# Autodesk Inventor assembly: Marco_triciclo
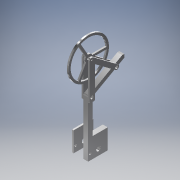
[picture p0: Inventor's stored thumbnail of the model, 180x180]
Saved by Autodesk Inventor 2019 (Build 230136000, 136)
## iProperties
Created: 2019-11-14
Part Number: Marco_triciclo
Document SubType Name: Assembly
Designer: Domenico
Mass: 2567.25 g
Surface Area: 2052.12 cm^2
Volume: 950.832 cm^3
Density: 2.7 g/cm^3
Author: Domenico
## Documents named in this file (5)
- C:\Users\Domenico\Documents\Inventor\Mecanismos2\Marco_triciclo.iam
- C:\Users\Domenico\Documents\Inventor\Mecanismos2\Marco_trasero_triciclo.ipt
- C:\Users\Domenico\Documents\Inventor\Mecanismos2\Marco_triciclo.ipt
- C:\Users\Domenico\Documents\Inventor\Mecanismos2\Marco_frontal.ipt
- C:\Users\Domenico\Documents\Inventor\Mecanismos2\Rueda_triciclo_trasera.ipt
## Components (5 placed, 4 different names)
1. Marco_trasero_triciclo:1 — Mate:1, Mate:2, Mate:3, Mate:13
2. Marco_triciclo:1 — Mate:1, Mate:2, Mate:3, Mate:4, Mate:5, Mate:6, Mate:9, Mate:10, Mate:11
3. Marco_trasero_triciclo:2 — Mate:4, Mate:5, Mate:6, Mate:12
4. Marco_frontal:1 — Mate:9, Mate:10, Mate:11
5. Rueda_triciclo_trasera:1 — Mate:12, Mate:13
## Relationships (11: Mate 11)
- Mate:1: Marco_trasero_triciclo:1 ↔ Marco_triciclo:1
- Mate:2: Marco_trasero_triciclo:1 ↔ Marco_triciclo:1
- Mate:3: Marco_trasero_triciclo:1 ↔ Marco_triciclo:1
- Mate:4: Marco_triciclo:1 ↔ Marco_trasero_triciclo:2
- Mate:5: Marco_triciclo:1 ↔ Marco_trasero_triciclo:2
- Mate:6: Marco_triciclo:1 ↔ Marco_trasero_triciclo:2
- Mate:9 (53.1 mm): Marco_triciclo:1 ↔ Marco_frontal:1
- Mate:10: Marco_triciclo:1 ↔ Marco_frontal:1
- Mate:11: Marco_triciclo:1 ↔ Marco_frontal:1
- Mate:12: Marco_trasero_triciclo:2 ↔ Rueda_triciclo_trasera:1
- Mate:13 (9 mm): Marco_trasero_triciclo:1 ↔ Rueda_triciclo_trasera:1
